# Autodesk Inventor assembly: Hoja oculta
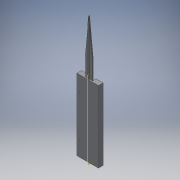
[picture p0: Inventor's stored thumbnail of the model, 180x180]
Saved by Autodesk Inventor 2016 (Build 200138000, 138)
## iProperties
Created: 2015-08-31
Part Number: Hoja oculta
Document SubType Name: Assembly
Designer: amatiasq
Author: amatiasq
## Documents named in this file (5)
- C:\Users\amatiasq\Documents\GitHub\3D\Hoja Oculta\Hoja oculta.iam
- C:\Users\amatiasq\Documents\GitHub\3D\Hoja Oculta\Base.ipt
- C:\Users\amatiasq\Documents\GitHub\3D\Hoja Oculta\Hoja.ipt
- C:\Users\amatiasq\Documents\GitHub\3D\Hoja Oculta\Tirador.ipt
- C:\Users\amatiasq\Documents\GitHub\3D\Hoja Oculta\Parametros.xlsx
## Components (4 placed, 3 different names)
1. Base:1 — Mate:1, Mate:2, Mate:3, Base-Tirador2, Base-Tirador1
2. Hoja:1 — Mate:1, Mate:2, Mate:3, Tirador2 Alto, Hoja-Tirador2, Tirador2 Lateral, Tirador1 Lateral, Tirador1 Alto, Hoja-Tirador1
3. Tirador:1 — Base-Tirador1, Tirador1 Lateral, Tirador1 Alto, Hoja-Tirador1
4. Tirador:2 — Base-Tirador2, Tirador2 Alto, Hoja-Tirador2, Tirador2 Lateral
## Relationships (11: Mate 11)
- Mate:1 (0.3 mm): Base:1 ↔ Hoja:1
- Mate:2: Base:1 ↔ Hoja:1
- Mate:3: Base:1 ↔ Hoja:1
- Base-Tirador2 [Mate]: Base:1 ↔ Tirador:2
- Tirador2 Alto [Mate] (0.3 mm): Hoja:1 ↔ Tirador:2
- Hoja-Tirador2 [Mate]: Hoja:1 ↔ Tirador:2
- Tirador2 Lateral [Mate] (0.3 mm): Hoja:1 ↔ Tirador:2
- Base-Tirador1 [Mate]: Base:1 ↔ Tirador:1
- Tirador1 Lateral [Mate] (0.3 mm): Hoja:1 ↔ Tirador:1
- Tirador1 Alto [Mate] (0.3 mm): Hoja:1 ↔ Tirador:1
- Hoja-Tirador1 [Mate]: Hoja:1 ↔ Tirador:1
## Named parameters: margen = 0.3 mm, base_largo = 200 mm, base_ancho = 60 mm, base_alto = 3 mm, muros_grosor = 3 mm, muros_alto = 10 mm, rail_alto = 1.5 mm, rail_grosor = 5 mm, hoja_ancho = 20 mm, hoja_largo = 200 mm, hoja_filo = 100 mm, hoja_stop_posicion = 5 mm, hoja_stop_saliente = 5 mm, hoja_stop_largo = 5 mm, hoja_alto = 3 mm, hoja_stop_biselado = 2 mm, hoja_filo_biselado = 0.5 mm, hoja_cola_biselado = 1 mm, hoja_ancho_total = 30 mm, soporte_deslizador_largo = 100 mm, soporte_deslizador_ancho = 5 mm, soporte_deslizador_alto = 5 mm, deslizador_soporte_ancho = 5 mm, deslizador_soporte_largo = 100 mm, deslizador_tope_alto = 5 mm, deslizador_soporte_alto = 5 mm, deslizador_tope_largo = 20 mm, deslizador_alto = 3 mm, tirador_agarre_largo = 3 mm, tirador_largo = 10 mm, movimiento_hoja = 100 mm
